# Autodesk Inventor assembly: 2 axis test stand
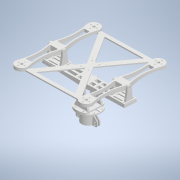
[picture p0: Inventor's stored thumbnail of the model, 180x180]
Saved by Autodesk Inventor 2020 (Build 240168000, 168)
## iProperties
Created: 2019-07-15
Part Number: 2 axis test stand
Document SubType Name: Assembly
Designer: Sean
Author: Sean
## Documents named in this file (6)
- C:\Users\Sean\Documents\Inventor\BalanceStand\2 axis test stand.iam
- C:\Users\Sean\Documents\Inventor\BalanceStand\HingePlate.ipt
- C:\Users\Sean\Documents\Inventor\BalanceStand\centerArm.iam
- C:\Users\Sean\Documents\Inventor\BalanceStand\LeverArm.ipt
- C:\Users\Sean\Documents\Inventor\BalanceStand\crossBraces.ipt
- C:\Users\Sean\Documents\Inventor\BalanceStand\MountingCollarFinal.ipt
## Components (7 placed, 5 different names)
1. HingePlate:1 — Insert:1, Insert:5, Insert:6
2. centerArm:1 [sub-assembly] — Insert:1, Insert:2, Insert:3
3. LeverArm:1 — Insert:2
4. LeverArm:2 — Insert:3
5. crossBraces:1 — Mate:1, Flush:1, Flush:2
6. crossBraces:2 — Mate:1, Flush:1, Flush:2
7. MountingCollarFinal:1 — Insert:5, Insert:6
## Relationships (8: Insert 5, Flush 2, Mate 1)
- Insert:1 (-36.576 mm): HingePlate:1 ↔ centerArm:1
- Insert:2 (-36.449 mm): centerArm:1 ↔ LeverArm:1
- Insert:3 (-36.449 mm): centerArm:1 ↔ LeverArm:2
- Mate:1: crossBraces:1 ↔ crossBraces:2
- Flush:1: crossBraces:1 ↔ crossBraces:2
- Flush:2: crossBraces:1 ↔ crossBraces:2
- Insert:5: HingePlate:1 ↔ MountingCollarFinal:1
- Insert:6: HingePlate:1 ↔ MountingCollarFinal:1
